# Autodesk Inventor assembly: glue-tests
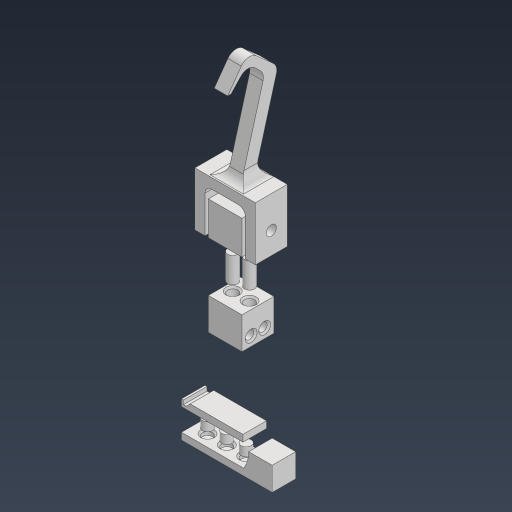
[picture p0: Inventor's stored thumbnail of the model, 512x512]
Saved by Autodesk Inventor 2023 (Build 270158000, 158)
## iProperties
Created: 2025-12-21
Part Number: glue-tests
Document SubType Name: Assembly
Designer: szymo
Author: szymo
## Documents named in this file (8)
- D:\tech\diy\e-skateboard\projekcik-inventor\other-parts\glue-tests.iam
- D:\tech\diy\e-skateboard\projekcik-inventor\glue_test_PULLING.ipt
- D:\tech\diy\e-skateboard\projekcik-inventor\other-parts\glue_test_PULLING_2.ipt
- D:\tech\diy\e-skateboard\projekcik-inventor\other-parts\glue_test_PULLING_pin.ipt
- D:\tech\diy\e-skateboard\projekcik-inventor\other-parts\glue_test_flex.ipt
- D:\tech\diy\e-skateboard\projekcik-inventor\other-parts\glue_test_flex_2.ipt
- D:\tech\diy\e-skateboard\projekcik-inventor\other-parts\glue_test_flex_pin.ipt
- D:\tech\diy\e-skateboard\projekcik-inventor\other-parts\steps\hook.ipt
## Components (10 placed, 7 different names)
1. glue_test_PULLING:1 — Flush:1, Flush:2, Mate:1, Mate:2
2. glue_test_PULLING_2:1 — Flush:1, Flush:2, Flush:5
3. glue_test_PULLING_pin:1 — Mate:1
4. glue_test_PULLING_pin:2 — Mate:2
5. glue_test_flex:1 — Mate:3, Mate:4, Mate:5, Flush:3, Flush:4
6. glue_test_flex_2:1 — Flush:3, Flush:4
7. glue_test_flex_pin:1 — Mate:3
8. glue_test_flex_pin:2 — Mate:4
9. glue_test_flex_pin:3 — Mate:5
10. hook:1 — Flush:5
## Relationships (10: Flush 5, Mate 5)
- Flush:1: glue_test_PULLING:1 ↔ glue_test_PULLING_2:1
- Flush:2: glue_test_PULLING:1 ↔ glue_test_PULLING_2:1
- Mate:1: glue_test_PULLING:1 ↔ glue_test_PULLING_pin:1
- Mate:2: glue_test_PULLING:1 ↔ glue_test_PULLING_pin:2
- Mate:3: glue_test_flex:1 ↔ glue_test_flex_pin:1
- Mate:4: glue_test_flex:1 ↔ glue_test_flex_pin:2
- Mate:5: glue_test_flex:1 ↔ glue_test_flex_pin:3
- Flush:3: glue_test_flex:1 ↔ glue_test_flex_2:1
- Flush:4: glue_test_flex:1 ↔ glue_test_flex_2:1
- Flush:5: glue_test_PULLING_2:1 ↔ hook:1
